# Autodesk Inventor assembly: Ball Screw Linear Actuator
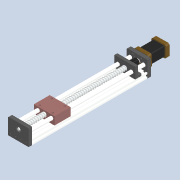
[picture p0: Inventor's stored thumbnail of the model, 180x180]
Saved by Autodesk Inventor 2022 (Build 260153000, 153)
## iProperties
Created: 2021-05-27
Part Number: Ball Screw Linear Actuator
Document SubType Name: Assembly
Designer: Coy
Author: Coy
Sending System: SolidWorks 2018
Last Author: USER
Last Saved: 2021-06-26
## Documents named in this file (12)
- H:\3D Files\Project 3D Models\Stock Parts\Linear Actuators\Ball Screw Linear Actuator.iam
- H:\3D Files\Downloaded 3D Files\GrabCad Downloads\linear-actuator-38.snapshot.1\rail.ipt
- H:\3D Files\Downloaded 3D Files\GrabCad Downloads\linear-actuator-38.snapshot.1\bottom plate.ipt
- H:\3D Files\Downloaded 3D Files\GrabCad Downloads\linear-actuator-38.snapshot.1\top plate modified.ipt
- H:\3D Files\Downloaded 3D Files\GrabCad Downloads\linear-actuator-38.snapshot.1\support column.ipt
- H:\3D Files\Downloaded 3D Files\GrabCad Downloads\linear-actuator-38.snapshot.1\holder.ipt
- H:\3D Files\Downloaded 3D Files\GrabCad Downloads\linear-actuator-38.snapshot.1\bearing.ipt
- H:\3D Files\Downloaded 3D Files\GrabCad Downloads\linear-actuator-38.snapshot.1\Part1^Linear actuator.ipt
- H:\3D Files\Downloaded 3D Files\GrabCad Downloads\linear-actuator-38.snapshot.1\thread.ipt
- H:\3D Files\Downloaded 3D Files\GrabCad Downloads\linear-actuator-38.snapshot.1\rotator.ipt
- H:\3D Files\Downloaded 3D Files\GrabCad Downloads\linear-actuator-38.snapshot.1\top.ipt
- H:\3D Files\Downloaded 3D Files\GrabCad Downloads\linear-actuator-38.snapshot.1\motor.ipt
## Components (13 placed, 11 different names)
1. rail:1
2. bottom plate:2 — Mate:1
3. top plate modified:1
4. support column:1
5. support column:2
6. holder:1
7. bearing:1
8. bearing:2
9. Part1^Linear actuator:1
10. thread:1
11. rotator:1
12. top:1 — Mate:1
13. motor:1
## Relationships (1: Mate 1)
- Mate:1 (200 mm): bottom plate:2 ↔ top:1
